# Autodesk Inventor assembly: Assembly2
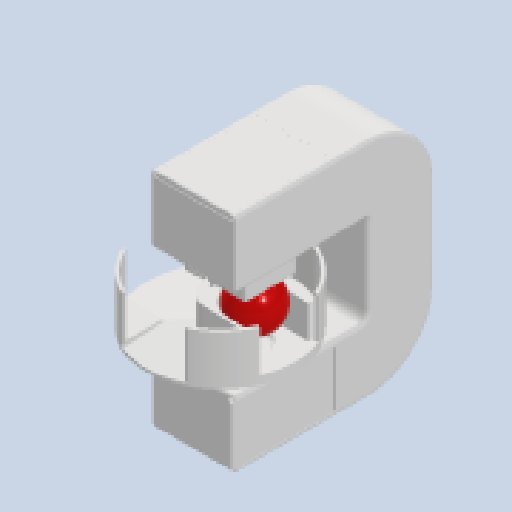
[picture p0: Inventor's stored thumbnail of the model, 512x512]
Saved by Autodesk Inventor 2025.4 (Build 294407000, 407)
## iProperties
Created: 2026-03-10
Part Number: Assembly2
Document SubType Name: Assembly
Designer: Amir
Author: Amir
## Documents named in this file (10)
- D:\basics project\Basics of Mechatronics (FINAAAAAL!!!!)\Basics of Mechatronics\Assembly2.iam
- D:\basics project\Basics of Mechatronics (FINAAAAAL!!!!)\Basics of Mechatronics\final pin.ipt
- D:\basics project\Basics of Mechatronics (FINAAAAAL!!!!)\Basics of Mechatronics\Parttt.ipt
- D:\basics project\Basics of Mechatronics (FINAAAAAL!!!!)\Basics of Mechatronics\Part1.ipt
- D:\basics project\Basics of Mechatronics (FINAAAAAL!!!!)\Basics of Mechatronics\upper cover.ipt
- D:\basics project\Basics of Mechatronics (FINAAAAAL!!!!)\Basics of Mechatronics\sorting base.ipt
- D:\basics project\Basics of Mechatronics (FINAAAAAL!!!!)\Basics of Mechatronics\final sorrting.ipt
- D:\basics project\Basics of Mechatronics (FINAAAAAL!!!!)\Basics of Mechatronics\SG90_Model_A.ipt
- D:\basics project\Basics of Mechatronics (FINAAAAAL!!!!)\Basics of Mechatronics\TCS3200 Color Sensor Module.ipt
- D:\basics project\Basics of Mechatronics (FINAAAAAL!!!!)\Basics of Mechatronics\upper coverr.ipt
## Components (9 placed, 9 different names)
1. Parttt:1 — Mate:19, Mate:20, Mate:26, Mate:29, Flush:1, Flush:2, Mate:31, Flush:3, Mate:34
2. Part1:1 — Mate:36
3. final pin:1 — Mate:21, Mate:22, Mate:23, Mate:25
4. sorting base:1 — Mate:19, Mate:20, Mate:21, Mate:22, Mate:35
5. final sorrting:1 — Mate:23, Mate:35, Mate:36
6. SG90_Model_A:4 — Mate:25, Mate:26
7. TCS3200 Color Sensor Module:4 — Mate:29
8. upper cover:1 — Flush:1, Flush:3, Mate:34
9. upper coverr:1 — Flush:2, Mate:31
## Relationships (15: Mate 12, Flush 3)
- Mate:19: Parttt:1 ↔ sorting base:1
- Mate:20: Parttt:1 ↔ sorting base:1
- Mate:21: final pin:1 ↔ sorting base:1
- Mate:22: final pin:1 ↔ sorting base:1
- Mate:23: final pin:1 ↔ final sorrting:1
- Mate:25: final pin:1 ↔ SG90_Model_A:4
- Mate:26: Parttt:1 ↔ SG90_Model_A:4
- Mate:29: Parttt:1 ↔ TCS3200 Color Sensor Module:4
- Flush:1: Parttt:1 ↔ upper cover:1
- Flush:2: Parttt:1 ↔ upper coverr:1
- Mate:31: Parttt:1 ↔ upper coverr:1
- Flush:3: Parttt:1 ↔ upper cover:1
- Mate:34: Parttt:1 ↔ upper cover:1
- Mate:35: sorting base:1 ↔ final sorrting:1
- Mate:36: Part1:1 ↔ final sorrting:1
## Named parameters: Finish1_Area = 28.2743, Finish1_Thickness = 0.05 mm
note: some values were not read from the file. Shown as the stored number, unit unknown: "Finish1_Area".
